# Autodesk Inventor assembly: arm
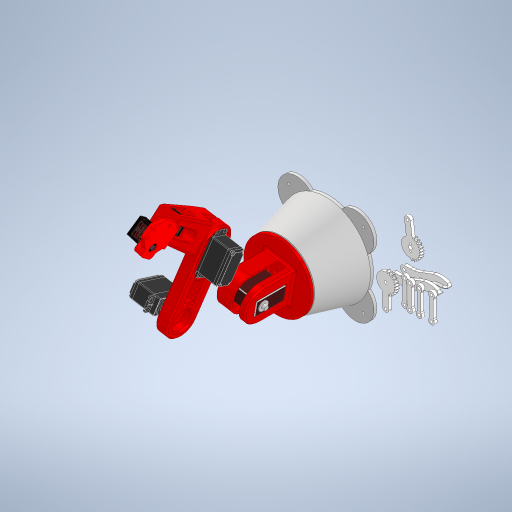
[picture p0: Inventor's stored thumbnail of the model, 512x512]
Saved by Autodesk Inventor 2023 (Build 270158000, 158)
## iProperties
Created: 2023-01-19
Part Number: arm
Document SubType Name: Assembly
Designer: denyh
Author: denyh
## Documents named in this file (14)
- C:\Users\denyh\Desktop\Rameno\arm.iam
- C:\Users\denyh\Desktop\Rameno\arm_base.ipt
- C:\Users\denyh\Desktop\Rameno\arm_base1.ipt
- C:\Users\denyh\Desktop\Rameno\Servo\MG_996R.iam
- C:\Users\denyh\Desktop\Rameno\arm_part2.ipt
- C:\Users\denyh\Desktop\Rameno\arm_part3.ipt
- C:\Users\denyh\Desktop\Rameno\lapak.ipt
- C:\Users\denyh\Desktop\Rameno\lapak2.ipt
- C:\Users\denyh\Desktop\Rameno\spojka.ipt
- C:\Users\denyh\Desktop\Rameno\zubate_kolo1.ipt
- C:\Users\denyh\Desktop\Rameno\zubate_kolo2.ipt
- C:\Users\denyh\Desktop\Rameno\grip_base.ipt
- C:\Users\denyh\Desktop\Rameno\Servo\SG90 Servo.ipt
- C:\Users\denyh\Desktop\Rameno\Servo\DualServo.ipt
## Components (19 placed, 13 different names)
1. arm_base:1 — Mate:1, Flush:1, Mate:17
2. arm_base1:1 — Rotational:1, Mate:14, Mate:15, Mate:16
3. MG_996R:1 [sub-assembly] — Mate:1, Flush:1, Rotational:1, Mate:17
4. arm_part2:1 — Rotational:2, Mate:5, Mate:6, Mate:7
5. arm_part3:1 — Rotational:3, Mate:8, Mate:9, Mate:10
6. lapak:1
7. lapak2:1
8. spojka:1
9. spojka:2
10. spojka:3
11. spojka:4
12. zubate_kolo1:1
13. zubate_kolo2:1
14. grip_base:1 — Rotational:4, Mate:11, Mate:12, Mate:13
15. MG_996R:2 [sub-assembly] — Mate:5, Mate:6, Mate:7, Rotational:3
16. MG_996R:4 [sub-assembly] — Rotational:2
17. SG90 Servo:1 — Mate:8, Mate:9, Mate:10, Rotational:4
18. SG90 Servo:2 — Mate:11, Mate:12, Mate:13
19. DualServo:1 — Mate:14, Mate:15, Mate:16
## Relationships (19: Mate 14, RevoluteJoint 4, Flush 1)
- Mate:1: arm_base:1 ↔ MG_996R:1
- Flush:1: arm_base:1 ↔ MG_996R:1
- Rotational:1 [RevoluteJoint]: arm_base1:1 ↔ MG_996R:1
- Rotational:2 [RevoluteJoint]: arm_part2:1 ↔ MG_996R:4
- Mate:5: arm_part2:1 ↔ MG_996R:2
- Mate:6 (0.5 mm): arm_part2:1 ↔ MG_996R:2
- Mate:7: arm_part2:1 ↔ MG_996R:2
- Rotational:3 [RevoluteJoint]: arm_part3:1 ↔ MG_996R:2
- Mate:8: arm_part3:1 ↔ SG90 Servo:1
- Mate:9 (0.5 mm): arm_part3:1 ↔ SG90 Servo:1
- Mate:10: arm_part3:1 ↔ SG90 Servo:1
- Rotational:4 [RevoluteJoint]: grip_base:1 ↔ SG90 Servo:1
- Mate:11: grip_base:1 ↔ SG90 Servo:2
- Mate:12: grip_base:1 ↔ SG90 Servo:2
- Mate:13 (0.5 mm): grip_base:1 ↔ SG90 Servo:2
- Mate:14: arm_base1:1 ↔ DualServo:1
- Mate:15: arm_base1:1 ↔ DualServo:1
- Mate:16: arm_base1:1 ↔ DualServo:1
- Mate:17: arm_base:1 ↔ MG_996R:1
